# Autodesk Inventor assembly: Camera_Assembly
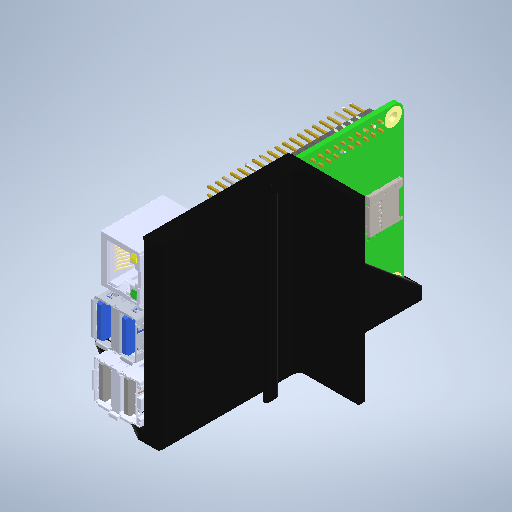
[picture p0: Inventor's stored thumbnail of the model, 512x512]
Saved by Autodesk Inventor 2025.1 (Build 291241000, 241)
## iProperties
Created: 2024-10-28
Part Number: Camera_Assembly
Document SubType Name: Assembly
Designer: Kai Altwicker
Author: Kai Altwicker
## iProperties of the stored document Raspberry Pi 4 Model B.ipt
Created: 2021-04-04
Part Number: Raspberry Pi 4 Model B
Material: Generisch
Document SubType Name: Modeling
Designer: Kai Altwicker
Density: 1 g/cm^3
Appearance: Vorgabe
Sending System: SolidWorks 2017
Last Author: Pieter Jan
Last Saved: 2021-04-04
Author: Kai Altwicker
## Documents named in this file (5)
- C:\Users\tallA\Repos\VolumanXR\hardware-capture\cad\rig_v2\Camera_Assembly.iam
- C:\Users\tallA\Repos\VolumanXR\hardware-capture\cad\rig_v2\VolumanXR_Rig_Cameraholder_v03.ipt
- **C:\Users\tallA\Repos\VolumanXR\hardware-capture\cad\rig_v2\Camera_Assembly.iam*LocalDocs*xAaaaaybaAaaaaaaaAaaaqx4pWg*Raspberry Pi 4 Model B.ipt
- C:\Users\tallA\Repos\VolumanXR\hardware-capture\cad\dimensions.xlsx
- C:\Users\tallA\Repos\VolumanXR\hardware-capture\cad\Library\Raspberry Pi 4 Model B.SLDPRT
## Components (2 placed, 2 different names)
1. VolumanXR_Rig_Cameraholder_v03:1 — Einfügen:1, Einfügen:2
2. Raspberry Pi 4 Model B:1 — Einfügen:1, Einfügen:2
## Relationships (2: Insert 2)
- Einfügen:1 [Insert]: VolumanXR_Rig_Cameraholder_v03:1 ↔ Raspberry Pi 4 Model B:1
- Einfügen:2 [Insert]: VolumanXR_Rig_Cameraholder_v03:1 ↔ Raspberry Pi 4 Model B:1
## Named parameters: d_tol = 0.3 mm, d_wand = 1.5 mm, l_profil_traeger = 1500 mm, l_profil_staender = 2500 mm, D_oct = 3621.32034 mm, h_profil_40x40 = 40 mm, b_profil_40x40 = 40 mm, h_profil_20x20 = 20 mm, b_profil_20x20 = 20 mm, d_traeger = 625 mm, l_profil_40x40 = 2500 mm, l_profil_20x20 = 1500 mm, D_hexadeca = 7541.00924 mm, l_rasp_pi = 85 mm, r_rasp_pi = 3 mm, b_rasp_pi = 56 mm
